# Autodesk Inventor assembly: ASM_Micron_OCT_Int
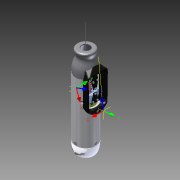
[picture p0: Inventor's stored thumbnail of the model, 180x180]
Saved by Autodesk Inventor 2011 SP2 (Build 150309200, 309)
## iProperties
Created: 2011-10-07
Part Number: ASM_Micron_OCT_Int
Document SubType Name: Assembly
Designer: sungwook
Author: sungwook
## Documents named in this file (19)
- C:\Users\sungwook\Documents\Inventor\Micron20_Base_Tube_Adjst\Assembly\OCT\ASM_Micron_OCT_Int.iam
- C:\Users\sungwook\Documents\Inventor\Micron20_Base_Tube_Adjst\Assembly\OCT\ASM_Micron_OCT_Probe.iam
- C:\Users\sungwook\Documents\Inventor\Micron20_Base_Tube_Adjst\Parts\ASAP\Handle_ASAP.iam
- C:\Users\sungwook\Documents\Inventor\Micron20_Base_Tube_Adjst\Parts\Electronics\PCB_Stack.iam
- C:\Users\sungwook\Documents\Inventor\Micron20_Base_Tube_Adjst\Parts\Handle\Handle_1_rev.ipt
- C:\Users\sungwook\Documents\Inventor\Micron20_Base_Tube_Adjst\Parts\Handle\Ver1(RP)\part\Handle_1_rev_Back.ipt
- C:\Users\sungwook\Documents\Inventor\Micron20_Base_Tube_Adjst\Parts\Handle\Ver1(RP)\Handle_1_rev_Back_part1.ipt
- C:\Users\sungwook\Documents\Inventor\Micron20_Base_Tube_Adjst\Parts\Handle\Ver1(RP)\Handle_1_rev_Back_part2.ipt
- C:\Users\sungwook\Documents\Inventor\Micron20_Base_Tube_Adjst\Parts\Handle\Window.ipt
- C:\Users\sungwook\Documents\Inventor\Micron20_Base_Tube_Adjst\Parts\Handle\Ver2(Al_RP)\Handle_2_Asm.iam
- C:\Users\sungwook\Documents\Inventor\Micron20_Base_Tube_Adjst\06082012_Outer_Tube\Outer_Tube.ipt
- C:\Users\sungwook\Documents\Inventor\Content Center Files\R2011\en-US\ANSI B18.6.3(00)\ANSI B18.6.3 - 0-80 UNF - 0.1875(32).ipt
- C:\Users\sungwook\Documents\Inventor\Micron20_Base_Tube_Adjst\Parts\Handle\Ver2(Al_RP)\Handle_2_Back_rev2.ipt
- C:\Users\sungwook\Documents\Inventor\Micron20_Base_Tube_Adjst\04192012_New_Front_2pcs\New_Front_Base_rev.ipt
- C:\Users\sungwook\Documents\Inventor\Micron20_Base_Tube_Adjst\04192012_New_Front_2pcs\New_Front_Upper_rev.ipt
- C:\Users\sungwook\Documents\Inventor\Micron20_Base_Tube_Adjst\04192012_New_Front_2pcs\New_Front_Upper_rev_v2.ipt
- C:\Users\sungwook\Documents\Inventor\Micron20_Base_Tube_Adjst\04192012_New_Front_2pcs\New_Front_Upper_rev_v3.ipt
- C:\Users\sungwook\Documents\Inventor\Content Center Files\R2011\en-US\ANSI B18.6.3(00)\ANSI B18.6.3 - 2-56 UNC - 0.1875(32).ipt
- C:\Users\sungwook\Documents\Inventor\Content Center Files\R2011\en-US\ANSI B18.6.3(00)\ANSI B18.6.3 - 2-56 UNC - 0.125(32).ipt
## Components (21 placed, 18 different names)
1. (0,0,0) [sub-assembly] — Mate:2, Mate:55, Mate:73, Mate:74, Mate:94, Mate:107, Mate:108
2. Handle_ASAP:1 [sub-assembly] — Mate:55
3. PCB_Stack:1 [sub-assembly] — Flush:73, Mate:73, Mate:74, Mate:103
4. New_Front_Base_rev:1 — Mate:112, Mate:113, Mate:114, Flush:74, Mate:120, Flush:121, Mate:121, Flush:123
5. New_Front_Upper_rev:1 — Mate:117, Flush:74, Mate:118, Mate:119
6. New_Front_Upper_rev_v2:1 — Mate:120, Flush:121, Flush:122, Mate:122
7. New_Front_Upper_rev_v3:1 — Mate:121, Flush:123, Flush:124
8. Cross Recessed 100° Flat Countersunk Head Machine Screw - Type I - Inch 2-56 UNC x 0.1875:1 — Mate:122
9. Cross Recessed 100° Flat Countersunk Head Machine Screw - Type I - Inch 2-56 UNC x 0.125:1 — Mate:123
10. Cross Recessed 100° Flat Countersunk Head Machine Screw - Type I - Inch 2-56 UNC x 0.125:2 — Mate:124
11. Window:1
12. Handle_1_rev_total — Mate:77, Mate:78
13. Handle_1_rev_Back:1
14. Handle_1_rev_Back_part1:1 — Mate:93, Mate:96
15. Handle_1_rev_Back_part2:1 — Mate:93, Mate:94, Mate:96
16. Handle_2_Asm:1 [sub-assembly] — Mate:101, Mate:102, Mate:103
17. Handle_2_Back_rev2:1 — Mate:109, Mate:110, Mate:111, Mate:123, Mate:124
18. Outer_Tube:1 — Mate:104, Mate:105, Mate:108, Mate:109, Mate:111, Mate:114, Mate:117, Mate:118, Mate:119, Flush:122, Flush:124
19. Cross Recessed 100° Flat Countersunk Head Machine Screw - Type I - Inch 0-80 UNF x 0.1875:1 — Mate:107
20. Cross Recessed 100° Flat Countersunk Head Machine Screw - Type I - Inch 0-80 UNF x 0.1875:2
21. Cross Recessed 100° Flat Countersunk Head Machine Screw - Type I - Inch 0-80 UNF x 0.1875:3
## Component patterns: (3 elements, first: Cross Recessed 100° Flat Countersunk Head Machine Screw - Type I - Inch 0-80 UNF x 0.1875:1)
## Relationships (36: Mate 30, Flush 6)
- Mate:2: (0,0,0)
- Mate:55: (0,0,0) ↔ Handle_ASAP:1
- Flush:73: PCB_Stack:1
- Mate:73: (0,0,0) ↔ PCB_Stack:1
- Mate:74: (0,0,0) ↔ PCB_Stack:1
- Mate:77: Handle_1_rev_total
- Mate:78: Handle_1_rev_total
- Mate:93: Handle_1_rev_Back_part1:1 ↔ Handle_1_rev_Back_part2:1
- Mate:94: (0,0,0) ↔ Handle_1_rev_Back_part2:1
- Mate:96: Handle_1_rev_Back_part1:1 ↔ Handle_1_rev_Back_part2:1
- Mate:101: Handle_2_Asm:1
- Mate:102: Handle_2_Asm:1
- Mate:103: PCB_Stack:1 ↔ Handle_2_Asm:1
- Mate:104: Outer_Tube:1
- Mate:105: Outer_Tube:1
- Mate:108: (0,0,0) ↔ Outer_Tube:1
- Mate:109: Handle_2_Back_rev2:1 ↔ Outer_Tube:1
- Mate:110: Handle_2_Back_rev2:1
- Mate:111: Handle_2_Back_rev2:1 ↔ Outer_Tube:1
- Mate:112: New_Front_Base_rev:1
- Mate:113: New_Front_Base_rev:1
- Mate:114: New_Front_Base_rev:1 ↔ Outer_Tube:1
- Mate:117: New_Front_Upper_rev:1 ↔ Outer_Tube:1
- Flush:74: New_Front_Base_rev:1 ↔ New_Front_Upper_rev:1
- Mate:118: New_Front_Upper_rev:1 ↔ Outer_Tube:1
- Mate:119: New_Front_Upper_rev:1 ↔ Outer_Tube:1
- Mate:120: New_Front_Base_rev:1 ↔ New_Front_Upper_rev_v2:1
- Flush:121: New_Front_Base_rev:1 ↔ New_Front_Upper_rev_v2:1
- Flush:122: New_Front_Upper_rev_v2:1 ↔ Outer_Tube:1
- Mate:121: New_Front_Base_rev:1 ↔ New_Front_Upper_rev_v3:1
- Flush:123: New_Front_Base_rev:1 ↔ New_Front_Upper_rev_v3:1
- Flush:124: New_Front_Upper_rev_v3:1 ↔ Outer_Tube:1
- Mate:107: (0,0,0) ↔ Cross Recessed 100° Flat Countersunk Head Machine Screw - Type I - Inch 0-80 UNF x 0.1875:1
- Mate:122: New_Front_Upper_rev_v2:1 ↔ Cross Recessed 100° Flat Countersunk Head Machine Screw - Type I - Inch 2-56 UNC x 0.1875:1
- Mate:123: Cross Recessed 100° Flat Countersunk Head Machine Screw - Type I - Inch 2-56 UNC x 0.125:1 ↔ Handle_2_Back_rev2:1
- Mate:124: Cross Recessed 100° Flat Countersunk Head Machine Screw - Type I - Inch 2-56 UNC x 0.125:2 ↔ Handle_2_Back_rev2:1
